# Autodesk Inventor assembly: Thumb_assembly_1
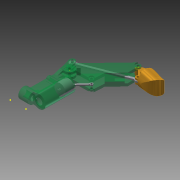
[picture p0: Inventor's stored thumbnail of the model, 180x180]
Saved by Autodesk Inventor 2015 (Build 190159000, 159)
## iProperties
Created: 2016-10-25
Part Number: Thumb_assembly_1
Document SubType Name: Assembly
Designer: Neelotpal Nag
Author: Neelotpal Nag
## Documents named in this file (8)
- D:\NEEL BACKUP\DISA 2016\Fingers 1\Thumb\Thumb_assembly_1.iam
- D:\NEEL BACKUP\DISA 2016\Fingers 1\Thumb\Thumb_Lower_main_1.ipt
- D:\NEEL BACKUP\DISA 2016\Fingers 1\Thumb\Thumb_Upper_main_1.ipt
- D:\NEEL BACKUP\DISA 2016\Fingers 1\Thumb\Thumb_Restrain_Pin_1.ipt
- D:\NEEL BACKUP\DISA 2016\Fingers 1\Thumb\ThumbNew_Base_Cylinder_11mm.ipt
- D:\NEEL BACKUP\DISA 2016\Fingers 1\Thumb\Cylinder_10.5mm.ipt
- D:\NEEL BACKUP\DISA 2016\Fingers 1\Thumb\Shaft_Piston.ipt
- D:\NEEL BACKUP\DISA 2016\Fingers 1\Thumb\Thumb_Shaft_Piston.ipt
## Components (7 placed, 7 different names)
1. Thumb_Lower_main_1:1 — Mate:3, Mate:4, Mate:7, Mate:9, Mate:11, Mate:15
2. Thumb_Upper_main_1:1 — Mate:3, Mate:4, Mate:6
3. Thumb_Restrain_Pin_1:1 — Mate:6, Mate:8, Mate:16
4. ThumbNew_Base_Cylinder_11mm:1 — Mate:7, Mate:8, Mate:9, Mate:10, Angle:1, Mate:16
5. Cylinder_10.5mm:1 — Mate:10, Angle:1, Mate:12, Mate:13, Mate:14
6. Shaft_Piston:1 — Mate:11, Mate:12
7. Thumb_Shaft_Piston:1 — Mate:13, Mate:14, Mate:15
## Relationships (14: Mate 13, Angle 1)
- Mate:3: Thumb_Lower_main_1:1 ↔ Thumb_Upper_main_1:1
- Mate:4 (0.5 mm): Thumb_Lower_main_1:1 ↔ Thumb_Upper_main_1:1
- Mate:6: Thumb_Upper_main_1:1 ↔ Thumb_Restrain_Pin_1:1
- Mate:7: Thumb_Lower_main_1:1 ↔ ThumbNew_Base_Cylinder_11mm:1
- Mate:8: Thumb_Restrain_Pin_1:1 ↔ ThumbNew_Base_Cylinder_11mm:1
- Mate:9: Thumb_Lower_main_1:1 ↔ ThumbNew_Base_Cylinder_11mm:1
- Mate:10: ThumbNew_Base_Cylinder_11mm:1 ↔ Cylinder_10.5mm:1
- Angle:1 (0 deg): ThumbNew_Base_Cylinder_11mm:1 ↔ Cylinder_10.5mm:1
- Mate:11: Thumb_Lower_main_1:1 ↔ Shaft_Piston:1
- Mate:12: Cylinder_10.5mm:1 ↔ Shaft_Piston:1
- Mate:13: Cylinder_10.5mm:1 ↔ Thumb_Shaft_Piston:1
- Mate:14: Cylinder_10.5mm:1 ↔ Thumb_Shaft_Piston:1
- Mate:15: Thumb_Lower_main_1:1 ↔ Thumb_Shaft_Piston:1
- Mate:16: Thumb_Restrain_Pin_1:1 ↔ ThumbNew_Base_Cylinder_11mm:1
